# Autodesk Inventor assembly: RasPiWCase
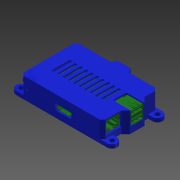
[picture p0: Inventor's stored thumbnail of the model, 180x180]
Saved by Autodesk Inventor 2015 (Build 190159000, 159)
## iProperties
Created: 2014-02-10
Part Number: RasPiWCase
Document SubType Name: Assembly
Designer: Jack
Author: Jack
## Documents named in this file (4)
- C:\Users\Jack\Sync\MendelMax1.5\InventorParts\Electronics\RasPiWCase.iam
- C:\Users\Jack\Sync\MendelMax1.5\InventorParts\Electronics\RaspiBbj.ipt
- C:\Users\Jack\Sync\MendelMax1.5\InventorParts\Electronics\RaspiCaseLower.ipt
- C:\Users\Jack\Sync\MendelMax1.5\InventorParts\Electronics\RaspiCaseUpper.ipt
## Components (3 placed, 3 different names)
1. RaspiBbj:1 — Mate:1, Mate:2, Mate:3
2. RaspiCaseLower:1 — Mate:1, Mate:2, Mate:3, Flush:1, Flush:2, Mate:4
3. RaspiCaseUpper:1 — Flush:1, Flush:2, Mate:4
## Relationships (6: Mate 4, Flush 2)
- Mate:1: RaspiBbj:1 ↔ RaspiCaseLower:1
- Mate:2 (0.5 mm): RaspiBbj:1 ↔ RaspiCaseLower:1
- Mate:3 (0.5 mm): RaspiBbj:1 ↔ RaspiCaseLower:1
- Flush:1: RaspiCaseLower:1 ↔ RaspiCaseUpper:1
- Flush:2: RaspiCaseLower:1 ↔ RaspiCaseUpper:1
- Mate:4: RaspiCaseLower:1 ↔ RaspiCaseUpper:1
